# Autodesk Inventor assembly: ASSEMBLY_Main
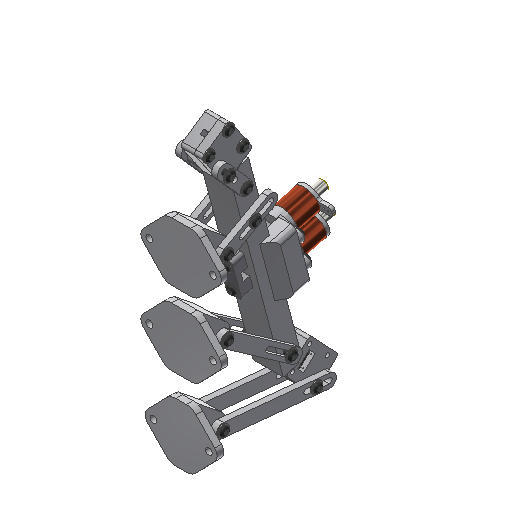
[picture p0: Inventor's stored thumbnail of the model, 512x512]
Saved by Autodesk Inventor 2026.1 (Build 301233000, 233)
## iProperties
Created: 2018-06-14
Part Number: ASSEMBLY_Main
Document SubType Name: Assembly
Designer: Andrzej
Author: Andrzej
## Documents named in this file (22)
- C:\Users\Andrzej\OneDrive\_DRIVE_SYNCH_FILES\__ BYTECHLAB PROJECTS\MLTDIS - Measurement Rail For SMD Parts\MCAD\1_REV1\ASSEMBLY_MAIN_REVA\ASSEMBLY_Main.iam
- C:\Users\Andrzej\OneDrive\_DRIVE_SYNCH_FILES\__ BYTECHLAB PROJECTS\MLTDIS - Measurement Rail For SMD Parts\MCAD\1_REV1\ASSEMBLY_MAIN_REVA\3DP_PLA_Measurement_Rail.ipt
- C:\Users\Andrzej\OneDrive\_DRIVE_SYNCH_FILES\__ BYTECHLAB PROJECTS\MLTDIS - Measurement Rail For SMD Parts\MCAD\1_REV1\ASSEMBLY_MAIN_REVA\ASSEMBLY_Solenoid_Actuator.iam
- C:\Users\Andrzej\OneDrive\_DRIVE_SYNCH_FILES\__ BYTECHLAB PROJECTS\MLTDIS - Measurement Rail For SMD Parts\MCAD\1_REV1\ASSEMBLY_MAIN_REVA\3DP_PLA_Measurement_Rail_Rammer.ipt
- C:\Users\Andrzej\OneDrive\_DRIVE_SYNCH_FILES\__ BYTECHLAB PROJECTS\MLTDIS - Measurement Rail For SMD Parts\MCAD\1_REV1\ASSEMBLY_MAIN_REVA\3DP_PLA_Measurement_Rail_Barrier.ipt
- C:\Users\Andrzej\OneDrive\_DRIVE_SYNCH_FILES\__ BYTECHLAB PROJECTS\MLTDIS - Measurement Rail For SMD Parts\MCAD\1_REV1\ASSEMBLY_MAIN_REVA\3DP_PLA_Measurement_Rail_Base.ipt
- C:\Users\Andrzej\OneDrive\_DRIVE_SYNCH_FILES\__ BYTECHLAB PROJECTS\MLTDIS - Measurement Rail For SMD Parts\MCAD\1_REV1\ASSEMBLY_MAIN_REVA\3DP_PLA_Measurement_Rail_Mounting_Bracket_Long.ipt
- C:\Users\Andrzej\OneDrive\_DRIVE_SYNCH_FILES\__ BYTECHLAB PROJECTS\MLTDIS - Measurement Rail For SMD Parts\MCAD\1_REV1\ASSEMBLY_MAIN_REVA\3DP_PLA_Measurement_Rail_Mounting_Bracket_Short.ipt
- C:\Users\Andrzej\OneDrive\_DRIVE_SYNCH_FILES\__ BYTECHLAB PROJECTS\MLTDIS - Measurement Rail For SMD Parts\MCAD\1_REV1\ASSEMBLY_MAIN_REVA\3DP_PLA_Measurement_Rail_Vibration_Motor_Clamp.ipt
- C:\Users\Andrzej\OneDrive\_DRIVE_SYNCH_FILES\__ BYTECHLAB PROJECTS\MLTDIS - Measurement Rail For SMD Parts\MCAD\1_REV1\ASSEMBLY_MAIN_REVA\CNCM_FR4_Measurement_Rail_Contacts.ipt
- C:\Users\Andrzej\OneDrive\_DRIVE_SYNCH_FILES\__ BYTECHLAB PROJECTS\MLTDIS - Measurement Rail For SMD Parts\MCAD\1_REV1\ASSEMBLY_MAIN_REVA\ASSEMBLY_Part_Detector.iam
- C:\Users\Andrzej\OneDrive\_DRIVE_SYNCH_FILES\__ BYTECHLAB PROJECTS\MLTDIS - Measurement Rail For SMD Parts\MCAD\1_REV1\ASSEMBLY_MAIN_REVA\3DP_PLA_Part_Detector_Base.ipt
- C:\Users\Andrzej\OneDrive\_DRIVE_SYNCH_FILES\__ BYTECHLAB PROJECTS\MLTDIS - Measurement Rail For SMD Parts\MCAD\1_REV1\ASSEMBLY_MAIN_REVA\3DP_PLA_Part_Detector_Mounting_Bracket.ipt
- C:\Users\Andrzej\OneDrive\_DRIVE_SYNCH_FILES\__ BYTECHLAB PROJECTS\MLTDIS - Measurement Rail For SMD Parts\MCAD\1_REV1\ASSEMBLY_MAIN_REVA\3DP_PLA_Part_Detector_Mounting_Bracket_Short.ipt
- C:\Users\Andrzej\OneDrive\_DRIVE_SYNCH_FILES\__ BYTECHLAB PROJECTS\MLTDIS - Measurement Rail For SMD Parts\MCAD\1_REV1\ASSEMBLY_MAIN_REVA\3DP_PLA_Part_Detector_Mounting_Bracket_Short_Washer.ipt
- C:\Users\Andrzej\OneDrive\_DRIVE_SYNCH_FILES\__ BYTECHLAB PROJECTS\MLTDIS - Measurement Rail For SMD Parts\MCAD\1_REV1\__CONTENT_CENTER_PARTS\en-US\DIN 125-2  A\DIN 125-2 - A 3,2A.ipt
- C:\Users\Andrzej\OneDrive\_DRIVE_SYNCH_FILES\__ BYTECHLAB PROJECTS\MLTDIS - Measurement Rail For SMD Parts\MCAD\1_REV1\__CONTENT_CENTER_PARTS\en-US\ISO 7380-1\ISO 7380-1 - M3 x 10.ipt
- C:\Users\Andrzej\OneDrive\_DRIVE_SYNCH_FILES\__ BYTECHLAB PROJECTS\MLTDIS - Measurement Rail For SMD Parts\MCAD\1_REV1\__CONTENT_CENTER_PARTS\en-US\ISO 7380-1\ISO 7380-1 - M3 x 8.ipt
- C:\Users\Andrzej\OneDrive\_DRIVE_SYNCH_FILES\__ BYTECHLAB PROJECTS\MLTDIS - Measurement Rail For SMD Parts\MCAD\1_REV1\__CONTENT_CENTER_PARTS\en-US\ISO 7380-1\ISO 7380-1 - M3 x 12.ipt
- C:\Users\Andrzej\OneDrive\_DRIVE_SYNCH_FILES\__ BYTECHLAB PROJECTS\MLTDIS - Measurement Rail For SMD Parts\MCAD\1_REV1\__CONTENT_CENTER_PARTS\en-US\ISO 7380-1\ISO 7380-1 - M3 x 25.ipt
- C:\Users\Andrzej\OneDrive\_DRIVE_SYNCH_FILES\__ BYTECHLAB PROJECTS\MLTDIS - Measurement Rail For SMD Parts\MCAD\1_REV1\__CONTENT_CENTER_PARTS\en-US\ISO 7380-1\ISO 7380-1 - M3 x 30.ipt
- C:\Users\Andrzej\OneDrive\_DRIVE_SYNCH_FILES\__ BYTECHLAB PROJECTS\MLTDIS - Measurement Rail For SMD Parts\MCAD\1_REV1\__CONTENT_CENTER_PARTS\en-US\DIN 934\DIN 934 - M3 x 0,5.ipt
## Components (77 placed, 21 different names)
1. 3DP_PLA_Measurement_Rail:1 — Mate:1, Mate:2, Mate:3, Mate:4, Mate:5, Mate:6, Flush:1, Flush:2, Angle:1, Mate:23, Mate:24, Mate:25, Mate:26, Mate:29, Mate:30, Mate:31, Mate:32, Mate:34, Mate:35, Mate:37, Mate:38, Mate:39, Mate:40, Flush:6, Mate:49, Mate:50, Mate:51, Mate:52, Mate:64, Mate:66, Mate:74, Mate:76
2. ASSEMBLY_Solenoid_Actuator:1 [sub-assembly] — Mate:2, Mate:3, Mate:4, Mate:36, Mate:80, Mate:81, Mate:83, Mate:84, Mate:85, Mate:87
3. ASSEMBLY_Solenoid_Actuator:2 [sub-assembly] — Mate:1, Mate:5, Mate:6, Mate:33, Mate:82, Mate:86
4. 3DP_PLA_Measurement_Rail_Rammer:1 — Mate:32, Mate:33, Mate:34
5. 3DP_PLA_Measurement_Rail_Barrier:1 — Mate:35, Mate:36, Mate:37
6. 3DP_PLA_Measurement_Rail_Base:1 — Flush:1, Mate:13, Mate:15, Mate:17, Mate:18, Flush:3, Flush:4, Flush:5
7. 3DP_PLA_Measurement_Rail_Base:2 — Flush:2, Flush:3, Angle:1, Mate:19, Mate:20, Mate:21, Mate:22, Mate:27, Mate:28
8. 3DP_PLA_Measurement_Rail_Mounting_Bracket_Long:1 — Mate:15, Mate:17, Mate:26, Mate:58
9. 3DP_PLA_Measurement_Rail_Mounting_Bracket_Long:4 — Mate:13, Mate:18, Mate:25, Mate:70
10. 3DP_PLA_Measurement_Rail_Mounting_Bracket_Short:1 — Mate:20, Mate:21, Mate:24, Mate:68, Mate:69, Mate:71, Mate:75, Mate:77, Mate:79
11. 3DP_PLA_Measurement_Rail_Mounting_Bracket_Short:2 — Mate:19, Mate:22, Mate:23, Mate:56, Mate:57, Mate:59, Mate:63, Mate:65, Mate:67
12. 3DP_PLA_Measurement_Rail_Vibration_Motor_Clamp:1 — Mate:29, Mate:30, Mate:31, Mate:88, Mate:89, Mate:90, Mate:91
13. CNCM_FR4_Measurement_Rail_Contacts:1 — Mate:38, Mate:39, Mate:40
14. ASSEMBLY_Part_Detector:1 [sub-assembly] — Mate:44, Mate:45, Mate:48, Insert:23, Insert:25, Insert:26, Mate:96, Mate:97
15. 3DP_PLA_Part_Detector_Base:1 — Flush:4, Flush:5, Mate:41, Mate:42, Mate:46, Mate:47
16. 3DP_PLA_Part_Detector_Mounting_Bracket:1 — Mate:41, Mate:42, Mate:44, Mate:45, Mate:72, Mate:95, Mate:73
17. 3DP_PLA_Part_Detector_Mounting_Bracket:2 — Mate:46, Mate:47, Mate:48, Mate:60, Mate:94, Mate:61
18. ASSEMBLY_Part_Detector:2 [sub-assembly] — Flush:6, Mate:53, Mate:54, Mate:55, Insert:19, Insert:20, Insert:22, Mate:98
19. 3DP_PLA_Part_Detector_Mounting_Bracket_Short:1 — Mate:49, Mate:50, Flush:7, Mate:53, Mate:62, Mate:92
20. 3DP_PLA_Part_Detector_Mounting_Bracket_Short:2 — Mate:51, Mate:52, Flush:7, Mate:78, Mate:93
21. 3DP_PLA_Part_Detector_Mounting_Bracket_Short_Washer:1 — Mate:54, Mate:55, Mate:99
22. DIN 125-2 A A 3,2:20 — Insert:20, Insert:28
23. DIN 125-2 A A 3,2:19 — Insert:19, Insert:27
24. ISO 7380-1 M3 x 12:2 — Insert:18
25. DIN 125-2 A A 3,2:18 — Mate:90, Mate:91, Insert:18
26. ISO 7380-1 M3 x 12:1 — Insert:17
27. DIN 125-2 A A 3,2:17 — Mate:88, Mate:89, Insert:17
28. ISO 7380-1 M3 x 8:4 — Insert:16
29. ISO 7380-1 M3 x 8:3 — Insert:15
30. ISO 7380-1 M3 x 8:2 — Insert:14
31. DIN 125-2 A A 3,2:16 — Mate:86, Mate:87, Insert:16
32. DIN 125-2 A A 3,2:15 — Mate:84, Mate:85, Insert:15
33. DIN 125-2 A A 3,2:14 — Mate:82, Mate:83, Insert:14
34. ISO 7380-1 M3 x 8:1 — Insert:13
35. DIN 125-2 A A 3,2:13 — Mate:80, Mate:81, Insert:13
36. ISO 7380-1 M3 x 10:12 — Insert:12
37. ISO 7380-1 M3 x 10:11 — Insert:11
38. ISO 7380-1 M3 x 10:10 — Insert:10
39. ISO 7380-1 M3 x 8:5 — Insert:9
40. ISO 7380-1 M3 x 10:8 — Insert:8
41. DIN 125-2 A A 3,2:12 — Mate:78, Mate:79, Insert:12
42. DIN 125-2 A A 3,2:11 — Mate:76, Mate:77, Insert:11
43. DIN 125-2 A A 3,2:10 — Mate:74, Mate:75, Insert:10
44. DIN 125-2 A A 3,2:9 — Mate:72, Mate:73, Insert:9
45. DIN 125-2 A A 3,2:8 — Mate:70, Mate:71, Insert:8
46. ISO 7380-1 M3 x 10:7 — Insert:7
47. DIN 125-2 A A 3,2:7 — Mate:68, Mate:69, Insert:7
48. ISO 7380-1 M3 x 10:6 — Insert:6
49. ISO 7380-1 M3 x 10:5 — Insert:5
50. ISO 7380-1 M3 x 10:4 — Insert:4
51. ISO 7380-1 M3 x 8:6 — Insert:3
52. ISO 7380-1 M3 x 10:2 — Insert:2
53. DIN 125-2 A A 3,2:6 — Mate:66, Mate:67, Insert:6
54. DIN 125-2 A A 3,2:5 — Mate:64, Mate:65, Insert:5
55. DIN 125-2 A A 3,2:4 — Mate:62, Mate:63, Insert:4
56. DIN 125-2 A A 3,2:3 — Mate:60, Mate:61, Insert:3
57. DIN 125-2 A A 3,2:2 — Mate:58, Mate:59, Insert:2
58. ISO 7380-1 M3 x 10:1 — Insert:1
59. DIN 125-2 A A 3,2:1 — Mate:56, Mate:57, Insert:1
60. DIN 934 - replaced by DIN EN 24032/28673/28674 M3:2 — Insert:35
61. DIN 934 - replaced by DIN EN 24032/28673/28674 M3:1 — Insert:34
62. ISO 7380-1 M3 x 25:1 — Mate:100, Mate:101
63. ISO 7380-1 M3 x 30:1 — Insert:33
64. DIN 125-2 A A 3,2:28 — Mate:94, Mate:97, Mate:100, Mate:101
65. DIN 125-2 A A 3,2:27 — Mate:95, Mate:96, Insert:34
66. DIN 125-2 A A 3,2:26 — Mate:93, Mate:99, Insert:35
67. DIN 125-2 A A 3,2:25 — Mate:92, Mate:98, Insert:33
68. ISO 7380-1 M3 x 12:8 — Insert:32
69. ISO 7380-1 M3 x 12:7 — Insert:31
70. ISO 7380-1 M3 x 12:6 — Insert:30
71. ISO 7380-1 M3 x 12:5 — Insert:29
72. ISO 7380-1 M3 x 12:4 — Insert:28
73. ISO 7380-1 M3 x 12:3 — Insert:27
74. DIN 125-2 A A 3,2:24 — Insert:26, Insert:31
75. DIN 125-2 A A 3,2:23 — Insert:25, Insert:30
76. DIN 125-2 A A 3,2:22 — Insert:23, Insert:32
77. DIN 125-2 A A 3,2:21 — Insert:22, Insert:29
## Relationships (133: Mate 92, Insert 33, Flush 7, Angle 1)
- Mate:1: 3DP_PLA_Measurement_Rail:1 ↔ ASSEMBLY_Solenoid_Actuator:2
- Mate:2: 3DP_PLA_Measurement_Rail:1 ↔ ASSEMBLY_Solenoid_Actuator:1
- Mate:3: 3DP_PLA_Measurement_Rail:1 ↔ ASSEMBLY_Solenoid_Actuator:1
- Mate:4: 3DP_PLA_Measurement_Rail:1 ↔ ASSEMBLY_Solenoid_Actuator:1
- Mate:5: 3DP_PLA_Measurement_Rail:1 ↔ ASSEMBLY_Solenoid_Actuator:2
- Mate:6: 3DP_PLA_Measurement_Rail:1 ↔ ASSEMBLY_Solenoid_Actuator:2
- Flush:1: 3DP_PLA_Measurement_Rail:1 ↔ 3DP_PLA_Measurement_Rail_Base:1
- Flush:2: 3DP_PLA_Measurement_Rail:1 ↔ 3DP_PLA_Measurement_Rail_Base:2
- Mate:13: 3DP_PLA_Measurement_Rail_Base:1 ↔ 3DP_PLA_Measurement_Rail_Mounting_Bracket_Long:4
- Mate:15: 3DP_PLA_Measurement_Rail_Base:1 ↔ 3DP_PLA_Measurement_Rail_Mounting_Bracket_Long:1
- Mate:17: 3DP_PLA_Measurement_Rail_Base:1 ↔ 3DP_PLA_Measurement_Rail_Mounting_Bracket_Long:1
- Mate:18: 3DP_PLA_Measurement_Rail_Base:1 ↔ 3DP_PLA_Measurement_Rail_Mounting_Bracket_Long:4
- Flush:3: 3DP_PLA_Measurement_Rail_Base:1 ↔ 3DP_PLA_Measurement_Rail_Base:2
- Angle:1 (-15 deg): 3DP_PLA_Measurement_Rail:1 ↔ 3DP_PLA_Measurement_Rail_Base:2
- Mate:19: 3DP_PLA_Measurement_Rail_Base:2 ↔ 3DP_PLA_Measurement_Rail_Mounting_Bracket_Short:2
- Mate:20: 3DP_PLA_Measurement_Rail_Base:2 ↔ 3DP_PLA_Measurement_Rail_Mounting_Bracket_Short:1
- Mate:21: 3DP_PLA_Measurement_Rail_Base:2 ↔ 3DP_PLA_Measurement_Rail_Mounting_Bracket_Short:1
- Mate:22: 3DP_PLA_Measurement_Rail_Base:2 ↔ 3DP_PLA_Measurement_Rail_Mounting_Bracket_Short:2
- Mate:23 (1.5 mm): 3DP_PLA_Measurement_Rail:1 ↔ 3DP_PLA_Measurement_Rail_Mounting_Bracket_Short:2
- Mate:24 (1.5 mm): 3DP_PLA_Measurement_Rail:1 ↔ 3DP_PLA_Measurement_Rail_Mounting_Bracket_Short:1
- Mate:25 (1.5 mm): 3DP_PLA_Measurement_Rail:1 ↔ 3DP_PLA_Measurement_Rail_Mounting_Bracket_Long:4
- Mate:26 (1.5 mm): 3DP_PLA_Measurement_Rail:1 ↔ 3DP_PLA_Measurement_Rail_Mounting_Bracket_Long:1
- Mate:27: 3DP_PLA_Measurement_Rail_Base:2
- Mate:28: 3DP_PLA_Measurement_Rail_Base:2
- Mate:29: 3DP_PLA_Measurement_Rail:1 ↔ 3DP_PLA_Measurement_Rail_Vibration_Motor_Clamp:1
- Mate:30: 3DP_PLA_Measurement_Rail:1 ↔ 3DP_PLA_Measurement_Rail_Vibration_Motor_Clamp:1
- Mate:31: 3DP_PLA_Measurement_Rail:1 ↔ 3DP_PLA_Measurement_Rail_Vibration_Motor_Clamp:1
- Mate:32 (0.5 mm): 3DP_PLA_Measurement_Rail:1 ↔ 3DP_PLA_Measurement_Rail_Rammer:1
- Mate:33: ASSEMBLY_Solenoid_Actuator:2 ↔ 3DP_PLA_Measurement_Rail_Rammer:1
- Mate:34: 3DP_PLA_Measurement_Rail:1 ↔ 3DP_PLA_Measurement_Rail_Rammer:1
- Mate:35 (0.5 mm): 3DP_PLA_Measurement_Rail:1 ↔ 3DP_PLA_Measurement_Rail_Barrier:1
- Mate:36: ASSEMBLY_Solenoid_Actuator:1 ↔ 3DP_PLA_Measurement_Rail_Barrier:1
- Mate:37: 3DP_PLA_Measurement_Rail:1 ↔ 3DP_PLA_Measurement_Rail_Barrier:1
- Mate:38: 3DP_PLA_Measurement_Rail:1 ↔ CNCM_FR4_Measurement_Rail_Contacts:1
- Mate:39: 3DP_PLA_Measurement_Rail:1 ↔ CNCM_FR4_Measurement_Rail_Contacts:1
- Mate:40: 3DP_PLA_Measurement_Rail:1 ↔ CNCM_FR4_Measurement_Rail_Contacts:1
- Flush:4: 3DP_PLA_Measurement_Rail_Base:1 ↔ 3DP_PLA_Part_Detector_Base:1
- Flush:5 (2.5 mm): 3DP_PLA_Measurement_Rail_Base:1 ↔ 3DP_PLA_Part_Detector_Base:1
- Mate:41: 3DP_PLA_Part_Detector_Base:1 ↔ 3DP_PLA_Part_Detector_Mounting_Bracket:1
- Mate:42: 3DP_PLA_Part_Detector_Base:1 ↔ 3DP_PLA_Part_Detector_Mounting_Bracket:1
- Mate:44: ASSEMBLY_Part_Detector:1 ↔ 3DP_PLA_Part_Detector_Mounting_Bracket:1
- Mate:45 (1.5 mm): ASSEMBLY_Part_Detector:1 ↔ 3DP_PLA_Part_Detector_Mounting_Bracket:1
- Mate:46: 3DP_PLA_Part_Detector_Base:1 ↔ 3DP_PLA_Part_Detector_Mounting_Bracket:2
- Mate:47: 3DP_PLA_Part_Detector_Base:1 ↔ 3DP_PLA_Part_Detector_Mounting_Bracket:2
- Mate:48 (1.5 mm): ASSEMBLY_Part_Detector:1 ↔ 3DP_PLA_Part_Detector_Mounting_Bracket:2
- Flush:6: 3DP_PLA_Measurement_Rail:1 ↔ ASSEMBLY_Part_Detector:2
- Mate:49: 3DP_PLA_Measurement_Rail:1 ↔ 3DP_PLA_Part_Detector_Mounting_Bracket_Short:1
- Mate:50: 3DP_PLA_Measurement_Rail:1 ↔ 3DP_PLA_Part_Detector_Mounting_Bracket_Short:1
- Mate:51: 3DP_PLA_Measurement_Rail:1 ↔ 3DP_PLA_Part_Detector_Mounting_Bracket_Short:2
- Mate:52: 3DP_PLA_Measurement_Rail:1 ↔ 3DP_PLA_Part_Detector_Mounting_Bracket_Short:2
- Flush:7: 3DP_PLA_Part_Detector_Mounting_Bracket_Short:1 ↔ 3DP_PLA_Part_Detector_Mounting_Bracket_Short:2
- Mate:53 (1.5 mm): ASSEMBLY_Part_Detector:2 ↔ 3DP_PLA_Part_Detector_Mounting_Bracket_Short:1
- Mate:54: ASSEMBLY_Part_Detector:2 ↔ 3DP_PLA_Part_Detector_Mounting_Bracket_Short_Washer:1
- Mate:55: ASSEMBLY_Part_Detector:2 ↔ 3DP_PLA_Part_Detector_Mounting_Bracket_Short_Washer:1
- Mate:56: 3DP_PLA_Measurement_Rail_Mounting_Bracket_Short:2 ↔ DIN 125-2 A A 3,2:1
- Mate:57: 3DP_PLA_Measurement_Rail_Mounting_Bracket_Short:2 ↔ DIN 125-2 A A 3,2:1
- Mate:58: 3DP_PLA_Measurement_Rail_Mounting_Bracket_Long:1 ↔ DIN 125-2 A A 3,2:2
- Mate:59: 3DP_PLA_Measurement_Rail_Mounting_Bracket_Short:2 ↔ DIN 125-2 A A 3,2:2
- Mate:60: 3DP_PLA_Part_Detector_Mounting_Bracket:2 ↔ DIN 125-2 A A 3,2:3
- Mate:61: 3DP_PLA_Part_Detector_Mounting_Bracket:2 ↔ DIN 125-2 A A 3,2:3
- Mate:62: 3DP_PLA_Part_Detector_Mounting_Bracket_Short:1 ↔ DIN 125-2 A A 3,2:4
- Mate:63: 3DP_PLA_Measurement_Rail_Mounting_Bracket_Short:2 ↔ DIN 125-2 A A 3,2:4
- Mate:64: 3DP_PLA_Measurement_Rail:1 ↔ DIN 125-2 A A 3,2:5
- Mate:65: 3DP_PLA_Measurement_Rail_Mounting_Bracket_Short:2 ↔ DIN 125-2 A A 3,2:5
- Mate:66: 3DP_PLA_Measurement_Rail:1 ↔ DIN 125-2 A A 3,2:6
- Mate:67: 3DP_PLA_Measurement_Rail_Mounting_Bracket_Short:2 ↔ DIN 125-2 A A 3,2:6
- Insert:1: ISO 7380-1 M3 x 10:1 ↔ DIN 125-2 A A 3,2:1
- Insert:2: ISO 7380-1 M3 x 10:2 ↔ DIN 125-2 A A 3,2:2
- Insert:3: ISO 7380-1 M3 x 8:6 ↔ DIN 125-2 A A 3,2:3
- Insert:4: ISO 7380-1 M3 x 10:4 ↔ DIN 125-2 A A 3,2:4
- Insert:5: ISO 7380-1 M3 x 10:5 ↔ DIN 125-2 A A 3,2:5
- Insert:6: ISO 7380-1 M3 x 10:6 ↔ DIN 125-2 A A 3,2:6
- Mate:68: 3DP_PLA_Measurement_Rail_Mounting_Bracket_Short:1 ↔ DIN 125-2 A A 3,2:7
- Mate:69: 3DP_PLA_Measurement_Rail_Mounting_Bracket_Short:1 ↔ DIN 125-2 A A 3,2:7
- Mate:70: 3DP_PLA_Measurement_Rail_Mounting_Bracket_Long:4 ↔ DIN 125-2 A A 3,2:8
- Mate:71: 3DP_PLA_Measurement_Rail_Mounting_Bracket_Short:1 ↔ DIN 125-2 A A 3,2:8
- Mate:72: 3DP_PLA_Part_Detector_Mounting_Bracket:1 ↔ DIN 125-2 A A 3,2:9
- Mate:73: 3DP_PLA_Part_Detector_Mounting_Bracket:1 ↔ DIN 125-2 A A 3,2:9
- Mate:74: 3DP_PLA_Measurement_Rail:1 ↔ DIN 125-2 A A 3,2:10
- Mate:75: 3DP_PLA_Measurement_Rail_Mounting_Bracket_Short:1 ↔ DIN 125-2 A A 3,2:10
- Mate:76: 3DP_PLA_Measurement_Rail:1 ↔ DIN 125-2 A A 3,2:11
- Mate:77: 3DP_PLA_Measurement_Rail_Mounting_Bracket_Short:1 ↔ DIN 125-2 A A 3,2:11
- Mate:78: 3DP_PLA_Part_Detector_Mounting_Bracket_Short:2 ↔ DIN 125-2 A A 3,2:12
- Mate:79: 3DP_PLA_Measurement_Rail_Mounting_Bracket_Short:1 ↔ DIN 125-2 A A 3,2:12
- Insert:7: ISO 7380-1 M3 x 10:7 ↔ DIN 125-2 A A 3,2:7
- Insert:8: ISO 7380-1 M3 x 10:8 ↔ DIN 125-2 A A 3,2:8
- Insert:9: ISO 7380-1 M3 x 8:5 ↔ DIN 125-2 A A 3,2:9
- Insert:10: ISO 7380-1 M3 x 10:10 ↔ DIN 125-2 A A 3,2:10
- Insert:11: ISO 7380-1 M3 x 10:11 ↔ DIN 125-2 A A 3,2:11
- Insert:12: ISO 7380-1 M3 x 10:12 ↔ DIN 125-2 A A 3,2:12
- Mate:80: ASSEMBLY_Solenoid_Actuator:1 ↔ DIN 125-2 A A 3,2:13
- Mate:81: ASSEMBLY_Solenoid_Actuator:1 ↔ DIN 125-2 A A 3,2:13
- Mate:82: ASSEMBLY_Solenoid_Actuator:2 ↔ DIN 125-2 A A 3,2:14
- Mate:83: ASSEMBLY_Solenoid_Actuator:1 ↔ DIN 125-2 A A 3,2:14
- Mate:84: ASSEMBLY_Solenoid_Actuator:1 ↔ DIN 125-2 A A 3,2:15
- Mate:85: ASSEMBLY_Solenoid_Actuator:1 ↔ DIN 125-2 A A 3,2:15
- Mate:86: ASSEMBLY_Solenoid_Actuator:2 ↔ DIN 125-2 A A 3,2:16
- Mate:87: ASSEMBLY_Solenoid_Actuator:1 ↔ DIN 125-2 A A 3,2:16
- Insert:13: ISO 7380-1 M3 x 8:1 ↔ DIN 125-2 A A 3,2:13
- Insert:14: ISO 7380-1 M3 x 8:2 ↔ DIN 125-2 A A 3,2:14
- Insert:15: ISO 7380-1 M3 x 8:3 ↔ DIN 125-2 A A 3,2:15
- Insert:16: ISO 7380-1 M3 x 8:4 ↔ DIN 125-2 A A 3,2:16
- Mate:88: 3DP_PLA_Measurement_Rail_Vibration_Motor_Clamp:1 ↔ DIN 125-2 A A 3,2:17
- Mate:89: 3DP_PLA_Measurement_Rail_Vibration_Motor_Clamp:1 ↔ DIN 125-2 A A 3,2:17
- Mate:90: 3DP_PLA_Measurement_Rail_Vibration_Motor_Clamp:1 ↔ DIN 125-2 A A 3,2:18
- Mate:91: 3DP_PLA_Measurement_Rail_Vibration_Motor_Clamp:1 ↔ DIN 125-2 A A 3,2:18
- Insert:17: ISO 7380-1 M3 x 12:1 ↔ DIN 125-2 A A 3,2:17
- Insert:18: ISO 7380-1 M3 x 12:2 ↔ DIN 125-2 A A 3,2:18
- Insert:19: ASSEMBLY_Part_Detector:2 ↔ DIN 125-2 A A 3,2:19
- Insert:20: ASSEMBLY_Part_Detector:2 ↔ DIN 125-2 A A 3,2:20
- Insert:22: ASSEMBLY_Part_Detector:2 ↔ DIN 125-2 A A 3,2:21
- Insert:23: ASSEMBLY_Part_Detector:1 ↔ DIN 125-2 A A 3,2:22
- Insert:25: ASSEMBLY_Part_Detector:1 ↔ DIN 125-2 A A 3,2:23
- Insert:26: ASSEMBLY_Part_Detector:1 ↔ DIN 125-2 A A 3,2:24
- Insert:27: DIN 125-2 A A 3,2:19 ↔ ISO 7380-1 M3 x 12:3
- Insert:28: DIN 125-2 A A 3,2:20 ↔ ISO 7380-1 M3 x 12:4
- Insert:29: ISO 7380-1 M3 x 12:5 ↔ DIN 125-2 A A 3,2:21
- Insert:30: ISO 7380-1 M3 x 12:6 ↔ DIN 125-2 A A 3,2:23
- Insert:31: ISO 7380-1 M3 x 12:7 ↔ DIN 125-2 A A 3,2:24
- Insert:32: ISO 7380-1 M3 x 12:8 ↔ DIN 125-2 A A 3,2:22
- Mate:92: 3DP_PLA_Part_Detector_Mounting_Bracket_Short:1 ↔ DIN 125-2 A A 3,2:25
- Mate:93: 3DP_PLA_Part_Detector_Mounting_Bracket_Short:2 ↔ DIN 125-2 A A 3,2:26
- Mate:94: 3DP_PLA_Part_Detector_Mounting_Bracket:2 ↔ DIN 125-2 A A 3,2:28
- Mate:95: 3DP_PLA_Part_Detector_Mounting_Bracket:1 ↔ DIN 125-2 A A 3,2:27
- Mate:96: ASSEMBLY_Part_Detector:1 ↔ DIN 125-2 A A 3,2:27
- Mate:97: ASSEMBLY_Part_Detector:1 ↔ DIN 125-2 A A 3,2:28
- Mate:98: ASSEMBLY_Part_Detector:2 ↔ DIN 125-2 A A 3,2:25
- Mate:99: 3DP_PLA_Part_Detector_Mounting_Bracket_Short_Washer:1 ↔ DIN 125-2 A A 3,2:26
- Insert:33: ISO 7380-1 M3 x 30:1 ↔ DIN 125-2 A A 3,2:25
- Mate:100: ISO 7380-1 M3 x 25:1 ↔ DIN 125-2 A A 3,2:28
- Mate:101: ISO 7380-1 M3 x 25:1 ↔ DIN 125-2 A A 3,2:28
- Insert:34: DIN 934 - replaced by DIN EN 24032/28673/28674 M3:1 ↔ DIN 125-2 A A 3,2:27
- Insert:35: DIN 934 - replaced by DIN EN 24032/28673/28674 M3:2 ↔ DIN 125-2 A A 3,2:26
